# Autodesk Inventor assembly: Assembly1
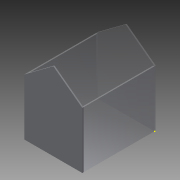
[picture p0: Inventor's stored thumbnail of the model, 180x180]
Saved by Autodesk Inventor 2015 (Build 190159000, 159)
## iProperties
Created: 2016-08-07
Part Number: Assembly1
Document SubType Name: Assembly
Designer: Gabriel
Author: Gabriel
## Documents named in this file (4)
- C:\Users\Gabriel\Desktop\TCC\Assembly1.iam
- C:\Users\Gabriel\Desktop\TCC\frente.ipt
- C:\Users\Gabriel\Desktop\TCC\fundo.ipt
- C:\Users\Gabriel\Desktop\TCC\lateral.ipt
## Components (4 placed, 3 different names)
1. frente:1 — Rotational:1, Rotational:2
2. fundo:1 — Rotational:3, Rotational:4, Planar:1
3. lateral:1 — Rotational:2, Rotational:4
4. lateral:2 — Rotational:1, Rotational:3, Planar:1
## Relationships (5: RevoluteJoint 4, PlanarJoint 1)
- Rotational:1 [RevoluteJoint]: frente:1 ↔ lateral:2
- Rotational:2 [RevoluteJoint]: frente:1 ↔ lateral:1
- Rotational:3 [RevoluteJoint]: fundo:1 ↔ lateral:2
- Rotational:4 [RevoluteJoint]: fundo:1 ↔ lateral:1
- Planar:1: fundo:1 ↔ lateral:2
